# Autodesk Inventor assembly: Case_Assembly
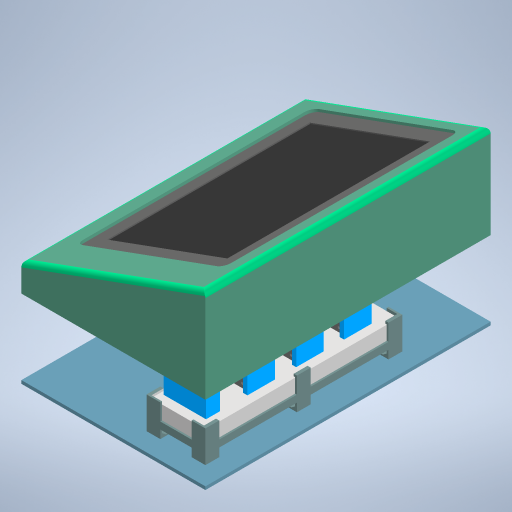
[picture p0: Inventor's stored thumbnail of the model, 512x512]
Saved by Autodesk Inventor 2024 (Build 280153000, 153)
## iProperties
Created: 2024-02-15
Part Number: Case_Assembly
Document SubType Name: Assembly
Designer: fabiancastano
Author: fabiancastano
## Documents named in this file (5)
- C:\GitHub\PulseLaserPrj\CaseDesign\Case_Assembly.iam
- C:\GitHub\PulseLaserPrj\CaseDesign\Polarizer.iam
- C:\GitHub\PulseLaserPrj\CaseDesign\Case_parts\BaseMotor.ipt
- C:\GitHub\PulseLaserPrj\CaseDesign\Case_parts\BaseCase.ipt
- C:\GitHub\PulseLaserPrj\CaseDesign\Case_parts\Screen_Case.iam
## Components (4 placed, 4 different names)
1. Polarizer:1 [sub-assembly] — Flush:1
2. BaseMotor:1 — Flush:1, Mate:1, Mate:2, Mate:3
3. BaseCase:1 — Mate:1, Mate:2, Mate:3, Flush:2, Flush:3
4. Screen_Case:1 [sub-assembly] — Flush:2, Flush:3
## Relationships (6: Flush 3, Mate 3)
- Flush:1: Polarizer:1 ↔ BaseMotor:1
- Mate:1: BaseMotor:1 ↔ BaseCase:1
- Mate:2: BaseMotor:1 ↔ BaseCase:1
- Mate:3: BaseMotor:1 ↔ BaseCase:1
- Flush:2: BaseCase:1 ↔ Screen_Case:1
- Flush:3: BaseCase:1 ↔ Screen_Case:1
